# Autodesk Inventor assembly: Tote Collector Arm_MIR
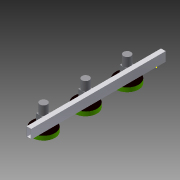
[picture p0: Inventor's stored thumbnail of the model, 180x180]
Saved by Autodesk Inventor 2015 (Build 190159000, 159)
## iProperties
Created: 2015-01-11
Part Number: Tote Collector Arm_MIR
Document SubType Name: Assembly
Designer: chapale16
Author: chapale16
## Documents named in this file (4)
- \\lhssvr02\Homedirs\Robotics Club\CAD Model 2015\Game Components\The Tote Collector-Arms\Tote Collector Arm_MIR.iam
- \\lhssvr02\Homedirs\Robotics Club\CAD Model 2015\Game Components\The Tote Collector-Arms\P60 Gear Box_MIR.ipt
- \\lhssvr02\Homedirs\Robotics Club\CAD Model 2015\Game Components\The Tote Collector-Arms\Arm_MIR.ipt
- \\lhssvr02\Homedirs\Robotics Club\CAD Model 2015\Game Components\The Tote Collector-Arms\collector arm wheel_MIR.ipt
## Components (7 placed, 3 different names)
1. P60 Gear Box_MIR:1 — Flush:5, Flush:1, Mate:4
2. P60 Gear Box_MIR:2 — Flush:6, Flush:2, Mate:5
3. P60 Gear Box_MIR:3 — Flush:4, Flush:3, Mate:6
4. Arm_MIR:1 — Flush:6, Flush:5, Flush:4
5. collector arm wheel_MIR:1 — Flush:3, Mate:6
6. collector arm wheel_MIR:2 — Flush:2, Mate:5
7. collector arm wheel_MIR:3 — Flush:1, Mate:4
## Relationships (9: Flush 6, Mate 3)
- Flush:6: P60 Gear Box_MIR:2 ↔ Arm_MIR:1
- Flush:5: P60 Gear Box_MIR:1 ↔ Arm_MIR:1
- Flush:4: P60 Gear Box_MIR:3 ↔ Arm_MIR:1
- Flush:3: P60 Gear Box_MIR:3 ↔ collector arm wheel_MIR:1
- Mate:6: P60 Gear Box_MIR:3 ↔ collector arm wheel_MIR:1
- Flush:2: P60 Gear Box_MIR:2 ↔ collector arm wheel_MIR:2
- Mate:5: P60 Gear Box_MIR:2 ↔ collector arm wheel_MIR:2
- Flush:1: P60 Gear Box_MIR:1 ↔ collector arm wheel_MIR:3
- Mate:4: P60 Gear Box_MIR:1 ↔ collector arm wheel_MIR:3
